# Autodesk Inventor assembly: Assembly3
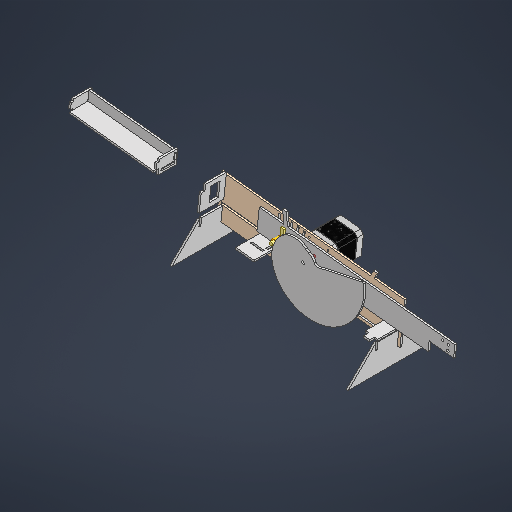
[picture p0: Inventor's stored thumbnail of the model, 512x512]
Saved by Autodesk Inventor 2027 (Build 310192000, 192)
## iProperties
Created: 2026-05-11
Part Number: Assembly3
Document SubType Name: Assembly
Designer: alexy
Author: alexy
## Documents named in this file (15)
- C:\Users\alexy\OneDrive\文件\group4\CarCourse_group4\SelfChosenTopic\Carinventor\3rdmodel\Assembly3-2.iam
- C:\Users\alexy\OneDrive\文件\group4\CarCourse_group4\SelfChosenTopic\Carinventor\3rdmodel\Sideboard3.ipt
- C:\Users\alexy\OneDrive\文件\group4\CarCourse_group4\SelfChosenTopic\Carinventor\3rdmodel\Nema 17 stepper motor.ipt
- C:\Users\alexy\OneDrive\文件\group4\CarCourse_group4\SelfChosenTopic\Carinventor\3rdmodel\Moving_rail3.ipt
- C:\Users\alexy\OneDrive\文件\group4\CarCourse_group4\SelfChosenTopic\Carinventor\3rdmodel\Frontrail.ipt
- C:\Users\alexy\OneDrive\文件\group4\CarCourse_group4\SelfChosenTopic\Carinventor\3rdmodel\Back_board.ipt
- C:\Users\alexy\OneDrive\文件\group4\CarCourse_group4\SelfChosenTopic\Carinventor\3rdmodel\Battary_holder.ipt
- C:\Users\alexy\OneDrive\文件\group4\CarCourse_group4\SelfChosenTopic\Carinventor\3rdmodel\Battary_holder_part2.ipt
- C:\Users\alexy\OneDrive\文件\group4\CarCourse_group4\SelfChosenTopic\Carinventor\3rdmodel\Battary_holder_part3.ipt
- C:\Users\alexy\OneDrive\文件\group4\CarCourse_group4\SelfChosenTopic\Carinventor\3rdmodel\contact_axis.ipt
- C:\Users\alexy\OneDrive\文件\group4\CarCourse_group4\SelfChosenTopic\Carinventor\3rdmodel\contact_axis_outer.ipt
- C:\Users\alexy\OneDrive\文件\group4\CarCourse_group4\SelfChosenTopic\Carinventor\3rdmodel\Middle_bar_hole.ipt
- C:\Users\alexy\OneDrive\文件\group4\CarCourse_group4\SelfChosenTopic\Carinventor\3rdmodel\Base.ipt
- C:\Users\alexy\OneDrive\文件\group4\CarCourse_group4\SelfChosenTopic\Carinventor\3rdmodel\Middle_bar_rect.ipt
- C:\Users\alexy\OneDrive\文件\group4\CarCourse_group4\SelfChosenTopic\Carinventor\3rdmodel\Cam_archi1.ipt
## Components (17 placed, 14 different names)
1. Sideboard3:1 — Mate:1, Insert:1, Mate:2, Mate:21, Mate:22, Mate:23, Mate:24, Mate:25, Mate:26, Flush:3, Flush:4, Mate:45, Mate:46, Mate:54, Mate:55, Mate:56, Mate:63, Angle:1, Mate:65, Mate:66, Mate:67
2. Nema 17 stepper motor:1 — Mate:1, Insert:1, Insert:4, Angle:1
3. Moving_rail3:1 — Mate:2, Mate:51, Mate:52, Mate:53, Mate:57, Mate:58, Mate:59
4. Sideboard3:3 — Flush:3, Flush:4, Mate:38
5. Frontrail:1 — Mate:21, Mate:22, Mate:23
6. Back_board:1 — Mate:24, Mate:25, Mate:26, Mate:38
7. Battary_holder:1 — Mate:42, Mate:43, Mate:44, Mate:45
8. Battary_holder:2 — Mate:35, Mate:36, Mate:37, Mate:39, Mate:40, Mate:41
9. Battary_holder_part2:1 — Mate:35, Mate:36, Mate:37, Mate:46
10. Battary_holder_part3:1 — Mate:39, Mate:40, Mate:41, Mate:42, Mate:43, Mate:44
11. contact_axis:1 — Insert:3, Mate:60, Mate:61, Mate:62
12. contact_axis_outer:1 — Insert:3
13. Middle_bar_hole:1 — Mate:51, Mate:52, Mate:53
14. Base:1 — Mate:54, Mate:55, Mate:56
15. Middle_bar_rect:1 — Mate:57, Mate:58, Mate:59, Mate:60, Mate:61, Mate:62, Mate:63
16. Cam_archi1:1 — Insert:4
17. Base:2 — Mate:65, Mate:66, Mate:67
## Relationships (42: Mate 36, Insert 3, Flush 2, Angle 1)
- Mate:1: Sideboard3:1 ↔ Nema 17 stepper motor:1
- Insert:1: Sideboard3:1 ↔ Nema 17 stepper motor:1
- Mate:2: Sideboard3:1 ↔ Moving_rail3:1
- Mate:21: Sideboard3:1 ↔ Frontrail:1
- Mate:22: Sideboard3:1 ↔ Frontrail:1
- Mate:23: Sideboard3:1 ↔ Frontrail:1
- Mate:24: Sideboard3:1 ↔ Back_board:1
- Mate:25: Sideboard3:1 ↔ Back_board:1
- Mate:26: Sideboard3:1 ↔ Back_board:1
- Flush:3: Sideboard3:1 ↔ Sideboard3:3
- Flush:4: Sideboard3:1 ↔ Sideboard3:3
- Mate:35: Battary_holder:2 ↔ Battary_holder_part2:1
- Mate:36: Battary_holder:2 ↔ Battary_holder_part2:1
- Mate:37: Battary_holder:2 ↔ Battary_holder_part2:1
- Mate:38: Sideboard3:3 ↔ Back_board:1
- Mate:39: Battary_holder:2 ↔ Battary_holder_part3:1
- Mate:40: Battary_holder:2 ↔ Battary_holder_part3:1
- Mate:41: Battary_holder:2 ↔ Battary_holder_part3:1
- Mate:42: Battary_holder:1 ↔ Battary_holder_part3:1
- Mate:43: Battary_holder:1 ↔ Battary_holder_part3:1
- Mate:44: Battary_holder:1 ↔ Battary_holder_part3:1
- Mate:45: Sideboard3:1 ↔ Battary_holder:1
- Mate:46: Sideboard3:1 ↔ Battary_holder_part2:1
- Insert:3 (5 mm): contact_axis:1 ↔ contact_axis_outer:1
- Mate:51: Moving_rail3:1 ↔ Middle_bar_hole:1
- Mate:52: Moving_rail3:1 ↔ Middle_bar_hole:1
- Mate:53: Moving_rail3:1 ↔ Middle_bar_hole:1
- Mate:54: Sideboard3:1 ↔ Base:1
- Mate:55: Sideboard3:1 ↔ Base:1
- Mate:56: Sideboard3:1 ↔ Base:1
- Mate:57: Moving_rail3:1 ↔ Middle_bar_rect:1
- Mate:58: Moving_rail3:1 ↔ Middle_bar_rect:1
- Mate:59: Moving_rail3:1 ↔ Middle_bar_rect:1
- Mate:60 (0.1 mm): contact_axis:1 ↔ Middle_bar_rect:1
- Mate:61: contact_axis:1 ↔ Middle_bar_rect:1
- Mate:62 (0.1 mm): contact_axis:1 ↔ Middle_bar_rect:1
- Mate:63 (2 mm): Sideboard3:1 ↔ Middle_bar_rect:1
- Insert:4: Nema 17 stepper motor:1 ↔ Cam_archi1:1
- Angle:1 (0 deg): Sideboard3:1 ↔ Nema 17 stepper motor:1
- Mate:65: Sideboard3:1 ↔ Base:2
- Mate:66: Sideboard3:1 ↔ Base:2
- Mate:67: Sideboard3:1 ↔ Base:2
